# Autodesk Inventor assembly: Cyl_Lens_Holder
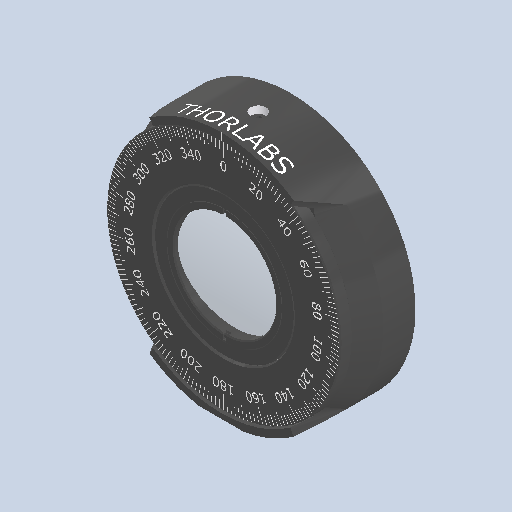
[picture p0: Inventor's stored thumbnail of the model, 512x512]
Saved by Autodesk Inventor 2024.2 (Build 282272000, 272)
## iProperties
Created: 2023-10-19
Part Number: Cyl_Lens_Holder
Document SubType Name: Assembly
Designer: S227943
Author: S227943
## Documents named in this file (3)
- C:\Users\monolithic\Documents\GitHub\CAD\Monolith\John\ASLM_SampleScanning_Baseplate\Assembly\Components\SubAssemblies\Cyl_Lens_Holder.iam
- C:\Users\monolithic\Documents\GitHub\CAD\Monolith\John\ASLM_SampleScanning_Baseplate\Assembly\Components\SubAssemblies\RSP1.ipt
- C:\Users\monolithic\Documents\GitHub\CAD\Monolith\John\ASLM_SampleScanning_Baseplate\Assembly\Components\SubAssemblies\ACY254-075-A-Step\ACY254-075-A-Step.ipt
## Components (2 placed, 2 different names)
1. RSP1:1 — Mate:1, Mate:2
2. ACY254-075-A-Step:1 — Mate:1, Mate:2
## Relationships (2: Mate 2)
- Mate:1: RSP1:1 ↔ ACY254-075-A-Step:1
- Mate:2: RSP1:1 ↔ ACY254-075-A-Step:1
